# Autodesk Inventor assembly: Cottini lamp2
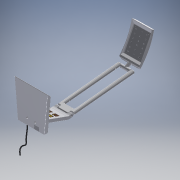
[picture p0: Inventor's stored thumbnail of the model, 180x180]
Saved by Autodesk Inventor 2016 (Build 200138000, 138)
## iProperties
Created: 2017-09-04
Part Number: Cottini lamp2
Document SubType Name: Assembly
Designer: Davide
Author: Davide
## Documents named in this file (25)
- C:\Users\Davide\Documents\Inventor\Lampetta\Lampetta.iam
- C:\Users\Davide\Documents\Inventor\Lampetta\base.ipt
- C:\Users\Davide\Documents\Inventor\Lampetta\rods_top-link.ipt
- C:\Users\Davide\Documents\Inventor\Lampetta\USB Case.ipt
- C:\Users\Davide\Documents\Inventor\Lampetta\cable.ipt
- C:\Users\Davide\Documents\Inventor\Lampetta\table.ipt
- C:\Users\Davide\Documents\Inventor\Lampetta\central_body.ipt
- C:\Users\Davide\Documents\Inventor\Lampetta\front_cover.ipt
- C:\Users\Davide\Documents\Inventor\Content Center Files\R2016\en-US\AS 1427(03)\AS 1427 - M2 x 5(1).ipt
- C:\Users\Davide\Documents\Inventor\Lampetta\Open_Book.ipt
- C:\Users\Davide\Documents\Inventor\Lampetta\projector.ipt
- C:\Users\Davide\Documents\Inventor\Lampetta\rods.ipt
- C:\Users\Davide\Documents\Inventor\Lampetta\rods_U-link.ipt
- C:\Users\Davide\Documents\Inventor\Content Center Files\R2016\en-US\AS 1112 (2)\AS 1112 - M4  Type 5.ipt
- C:\Users\Davide\Documents\Inventor\Content Center Files\R2016\en-US\AS 1427(05)\AS 1427 - M4 x 25(5) II.ipt
- C:\Users\Davide\Documents\Inventor\Content Center Files\R2016\en-US\AS 1420\AS 1420 - 1973 - M4 x 25.ipt
- C:\Users\Davide\Documents\Inventor\Content Center Files\R2016\en-US\AS 1112 (4)\AS 1112 - M4(2).ipt
- C:\Users\Davide\Documents\Inventor\Lampetta\button1.ipt
- C:\Users\Davide\Documents\Inventor\Lampetta\button2.ipt
- C:\Users\Davide\Documents\Inventor\Lampetta\button3.ipt
- C:\Users\Davide\Documents\Inventor\Lampetta\button4.ipt
- C:\Users\Davide\Documents\Inventor\Lampetta\USB-bay_cover.ipt
- C:\Users\Davide\Documents\Inventor\Lampetta\led_cover.ipt
- C:\Users\Davide\Documents\Inventor\Content Center Files\R2016\en-US\ANSI B18.6.5M(22)\ANSI B18.6.5M - M2x0,4 x 6(38).ipt
- C:\Users\Davide\Documents\Inventor\Lampetta\neopixel_6xled_strip.iam
## Components (42 placed, 24 different names)
1. base:1 — Mate:47, Mate:49, Mate:50, Mate:51, Mate:79, Flush:1, Mate:80, Mate:94, Mate:95, Mate:96, Mate:110, Mate:112, Mate:209, Mate:210, Mate:211
2. rods_top-link:1 — Mate:147, Mate:148, Mate:153, Mate:173, Mate:175, Mate:178, Mate:180, Mate:182, Mate:183
3. USB Case:1 — Mate:79, Flush:1, Mate:80
4. cable:1 — Mate:112
5. table:1 — Mate:94, Mate:146
6. central_body:1 — Mate:95, Mate:96, Mate:138, Mate:139, Mate:155, Mate:160, Mate:161, Mate:164, Mate:165, Mate:166, Mate:167, Mate:188, Mate:207, Mate:208
7. front_cover:1 — Flush:6, Flush:7, Mate:192, Flush:12, Mate:199, Mate:200, Flush:13, Mate:201, Mate:202, Flush:14, Mate:203, Mate:204, Flush:15, Mate:205, Mate:206, Mate:207, Mate:208
8. Open_Book:1 — Mate:146
9. projector:1 — Mate:147, Mate:148, Mate:214, Mate:215
10. rods:1 — Mate:149, Mate:150, Mate:151, Mate:153, Mate:169, Mate:170, Mate:171, Mate:172
11. rods_U-link:1 — Mate:149, Mate:150, Mate:151, Mate:155, Mate:168, Mate:185, Mate:187
12. button1:1 — Flush:12, Mate:199, Mate:200
13. button2:1 — Flush:13, Mate:201, Mate:202
14. button3:1 — Flush:14, Mate:203, Mate:204
15. button4:1 — Flush:15, Mate:205, Mate:206
16. USB-bay_cover:1 — Mate:209, Mate:210, Mate:211, Mate:212, Mate:213, Flush:16, Flush:17
17. led_cover:1 — Mate:214, Mate:215, Mate:216, Mate:217, Mate:218, Mate:219, Mate:220, Mate:221, Mate:222, Mate:223, Mate:226, Flush:18, Mate:227, Flush:19, Mate:228, Mate:229, Flush:20, Mate:230, Mate:231
18. neopixel_6xled_strip:1 [sub-assembly] — Mate:226, Flush:18, Mate:227
19. neopixel_6xled_strip:2 [sub-assembly] — Flush:20, Mate:230, Mate:231
20. neopixel_6xled_strip:3 [sub-assembly] — Flush:19, Mate:228, Mate:229
21. AS 1427 H - Metric M4 x 25:1 — Mate:47, Mate:51, Mate:158
22. AS 1427 H - Metric M4 x 25:2 — Mate:49, Mate:50, Mate:159
23. AS 1427 - Metric M2 x 5:2 — Mate:138, Flush:6, Mate:192
24. AS 1427 - Metric M2 x 5:3 — Mate:188
25. AS 1427 - Metric M2 x 5:6 — Mate:213, Flush:16
26. AS 1427 - Metric M2 x 5:7 — Mate:212, Flush:17
27. AS 1112 (2) - Metric M4  Type 5:1 — Mate:158, Mate:161
28. AS 1112 (2) - Metric M4  Type 5:2 — Mate:159, Mate:160
29. AS 1427 - Metric M2 x 5:4
30. AS 1427 - Metric M2 x 5:5 — Mate:139, Flush:7
31. AS 1420 - Metric M4 x 25:1 — Mate:164, Mate:167, Mate:184
32. AS 1420 - Metric M4 x 25:2 — Mate:165, Mate:166, Mate:168, Mate:186
33. AS 1420 - Metric M4 x 25:3 — Mate:169, Mate:170, Mate:175, Mate:178, Mate:179
34. AS 1420 - Metric M4 x 25:4 — Mate:171, Mate:172, Mate:173, Mate:181, Mate:182
35. AS 1112 (4) - Metric M4:1 — Mate:179, Mate:180
36. AS 1112 (4) - Metric M4:2 — Mate:181, Mate:183
37. AS 1112 (4) - Metric M4:3 — Mate:184, Mate:185
38. AS 1112 (4) - Metric M4:4 — Mate:186, Mate:187
39. Cross Recessed Pan Head Tapping Screw - Type D - Type I - Metric M2x0,4 x 6:1 — Mate:216, Mate:217
40. Cross Recessed Pan Head Tapping Screw - Type D - Type I - Metric M2x0,4 x 6:2 — Mate:218, Mate:219
41. Cross Recessed Pan Head Tapping Screw - Type D - Type I - Metric M2x0,4 x 6:3 — Mate:220, Mate:221
42. Cross Recessed Pan Head Tapping Screw - Type D - Type I - Metric M2x0,4 x 6:4 — Mate:222, Mate:223
## Relationships (93: Mate 81, Flush 12)
- Mate:47: base:1 ↔ AS 1427 H - Metric M4 x 25:1
- Mate:49: base:1 ↔ AS 1427 H - Metric M4 x 25:2
- Mate:50: base:1 ↔ AS 1427 H - Metric M4 x 25:2
- Mate:51: base:1 ↔ AS 1427 H - Metric M4 x 25:1
- Mate:79: base:1 ↔ USB Case:1
- Flush:1 (1 mm): base:1 ↔ USB Case:1
- Mate:80: base:1 ↔ USB Case:1
- Mate:94: base:1 ↔ table:1
- Mate:95: base:1 ↔ central_body:1
- Mate:96: base:1 ↔ central_body:1
- Mate:110: base:1
- Mate:112: base:1 ↔ cable:1
- Mate:138: central_body:1 ↔ AS 1427 - Metric M2 x 5:2
- Mate:139: central_body:1 ↔ AS 1427 - Metric M2 x 5:5
- Flush:6: front_cover:1 ↔ AS 1427 - Metric M2 x 5:2
- Flush:7: front_cover:1 ↔ AS 1427 - Metric M2 x 5:5
- Mate:146: table:1 ↔ Open_Book:1
- Mate:147: rods_top-link:1 ↔ projector:1
- Mate:148: rods_top-link:1 ↔ projector:1
- Mate:149: rods:1 ↔ rods_U-link:1
- Mate:150: rods:1 ↔ rods_U-link:1
- Mate:151: rods:1 ↔ rods_U-link:1
- Mate:153: rods_top-link:1 ↔ rods:1
- Mate:155: central_body:1 ↔ rods_U-link:1
- Mate:158: AS 1427 H - Metric M4 x 25:1 ↔ AS 1112 (2) - Metric M4  Type 5:1
- Mate:159: AS 1427 H - Metric M4 x 25:2 ↔ AS 1112 (2) - Metric M4  Type 5:2
- Mate:160: central_body:1 ↔ AS 1112 (2) - Metric M4  Type 5:2
- Mate:161: central_body:1 ↔ AS 1112 (2) - Metric M4  Type 5:1
- Mate:164: central_body:1 ↔ AS 1420 - Metric M4 x 25:1
- Mate:165: central_body:1 ↔ AS 1420 - Metric M4 x 25:2
- Mate:166 (-4 mm): central_body:1 ↔ AS 1420 - Metric M4 x 25:2
- Mate:167 (-4 mm): central_body:1 ↔ AS 1420 - Metric M4 x 25:1
- Mate:168: rods_U-link:1 ↔ AS 1420 - Metric M4 x 25:2
- Mate:169: rods:1 ↔ AS 1420 - Metric M4 x 25:3
- Mate:170 (-4 mm): rods:1 ↔ AS 1420 - Metric M4 x 25:3
- Mate:171: rods:1 ↔ AS 1420 - Metric M4 x 25:4
- Mate:172 (-4 mm): rods:1 ↔ AS 1420 - Metric M4 x 25:4
- Mate:173: rods_top-link:1 ↔ AS 1420 - Metric M4 x 25:4
- Mate:175: rods_top-link:1 ↔ AS 1420 - Metric M4 x 25:3
- [Mate]: AS 1420 - Metric M4 x 25:4 ↔ AS 1112 (4) - Metric M4:2
- [Mate]: rods_top-link:1 ↔ AS 1112 (4) - Metric M4:2
- Mate:178: rods_top-link:1 ↔ AS 1420 - Metric M4 x 25:3
- Mate:179: AS 1420 - Metric M4 x 25:3 ↔ AS 1112 (4) - Metric M4:1
- Mate:180: rods_top-link:1 ↔ AS 1112 (4) - Metric M4:1
- Mate:181: AS 1420 - Metric M4 x 25:4 ↔ AS 1112 (4) - Metric M4:2
- Mate:182: rods_top-link:1 ↔ AS 1420 - Metric M4 x 25:4
- Mate:183: rods_top-link:1 ↔ AS 1112 (4) - Metric M4:2
- Mate:184: AS 1420 - Metric M4 x 25:1 ↔ AS 1112 (4) - Metric M4:3
- Mate:185: rods_U-link:1 ↔ AS 1112 (4) - Metric M4:3
- Mate:186: AS 1420 - Metric M4 x 25:2 ↔ AS 1112 (4) - Metric M4:4
- Mate:187: rods_U-link:1 ↔ AS 1112 (4) - Metric M4:4
- Mate:188: central_body:1 ↔ AS 1427 - Metric M2 x 5:3
- Mate:192: front_cover:1 ↔ AS 1427 - Metric M2 x 5:2
- Flush:12: front_cover:1 ↔ button1:1
- Mate:199: front_cover:1 ↔ button1:1
- Mate:200: front_cover:1 ↔ button1:1
- Flush:13: front_cover:1 ↔ button2:1
- Mate:201: front_cover:1 ↔ button2:1
- Mate:202: front_cover:1 ↔ button2:1
- Flush:14: front_cover:1 ↔ button3:1
- Mate:203: front_cover:1 ↔ button3:1
- Mate:204: front_cover:1 ↔ button3:1
- Flush:15: front_cover:1 ↔ button4:1
- Mate:205: front_cover:1 ↔ button4:1
- Mate:206: front_cover:1 ↔ button4:1
- Mate:207: central_body:1 ↔ front_cover:1
- Mate:208: central_body:1 ↔ front_cover:1
- Mate:209: base:1 ↔ USB-bay_cover:1
- Mate:210: base:1 ↔ USB-bay_cover:1
- Mate:211: base:1 ↔ USB-bay_cover:1
- Mate:212: USB-bay_cover:1 ↔ AS 1427 - Metric M2 x 5:7
- Mate:213: USB-bay_cover:1 ↔ AS 1427 - Metric M2 x 5:6
- Flush:16: USB-bay_cover:1 ↔ AS 1427 - Metric M2 x 5:6
- Flush:17: USB-bay_cover:1 ↔ AS 1427 - Metric M2 x 5:7
- Mate:214: projector:1 ↔ led_cover:1
- Mate:215: projector:1 ↔ led_cover:1
- Mate:216: led_cover:1 ↔ Cross Recessed Pan Head Tapping Screw - Type D - Type I - Metric M2x0,4 x 6:1
- Mate:217: led_cover:1 ↔ Cross Recessed Pan Head Tapping Screw - Type D - Type I - Metric M2x0,4 x 6:1
- Mate:218: led_cover:1 ↔ Cross Recessed Pan Head Tapping Screw - Type D - Type I - Metric M2x0,4 x 6:2
- Mate:219: led_cover:1 ↔ Cross Recessed Pan Head Tapping Screw - Type D - Type I - Metric M2x0,4 x 6:2
- Mate:220: led_cover:1 ↔ Cross Recessed Pan Head Tapping Screw - Type D - Type I - Metric M2x0,4 x 6:3
- Mate:221: led_cover:1 ↔ Cross Recessed Pan Head Tapping Screw - Type D - Type I - Metric M2x0,4 x 6:3
- Mate:222: led_cover:1 ↔ Cross Recessed Pan Head Tapping Screw - Type D - Type I - Metric M2x0,4 x 6:4
- Mate:223: led_cover:1 ↔ Cross Recessed Pan Head Tapping Screw - Type D - Type I - Metric M2x0,4 x 6:4
- Mate:226: led_cover:1 ↔ neopixel_6xled_strip:1
- Flush:18: led_cover:1 ↔ neopixel_6xled_strip:1
- Mate:227: led_cover:1 ↔ neopixel_6xled_strip:1
- Flush:19: led_cover:1 ↔ neopixel_6xled_strip:3
- Mate:228: led_cover:1 ↔ neopixel_6xled_strip:3
- Mate:229: led_cover:1 ↔ neopixel_6xled_strip:3
- Flush:20: led_cover:1 ↔ neopixel_6xled_strip:2
- Mate:230: led_cover:1 ↔ neopixel_6xled_strip:2
- Mate:231: led_cover:1 ↔ neopixel_6xled_strip:2
